# Autodesk Inventor assembly: Stepper_with_Bracket
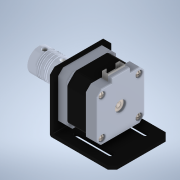
[picture p0: Inventor's stored thumbnail of the model, 180x180]
Saved by Autodesk Inventor 2020 (Build 240168000, 168)
## iProperties
Created: 2020-07-31
Part Number: Stepper_with_Bracket
Document SubType Name: Assembly
Designer: Abbas
Author: Abbas
## Documents named in this file (4)
- C:\Users\LENOVO\Desktop\Graduation Project\Fish Farming Unit\Feeding Mechanism\Stepper_with_Bracket.iam
- C:\Users\LENOVO\Desktop\Graduation Project\Fish Farming Unit\Feeding Mechanism\Stepper_Bracket.ipt
- C:\Users\LENOVO\Desktop\Graduation Project\Fish Farming Unit\Feeding Mechanism\Stepper_Motor.ipt
- C:\Users\LENOVO\Desktop\Graduation Project\Fish Farming Unit\Feeding Mechanism\NEMA17_Coupler.ipt
## Components (3 placed, 3 different names)
1. Stepper_Bracket:2 — Insert:1
2. Stepper_Motor:1 — Insert:1, Insert:2
3. NEMA17_Coupler:2 — Insert:2
## Relationships (2: Insert 2)
- Insert:1: Stepper_Bracket:2 ↔ Stepper_Motor:1
- Insert:2 (-10 mm): Stepper_Motor:1 ↔ NEMA17_Coupler:2
